# Autodesk Inventor assembly: Left Wheel
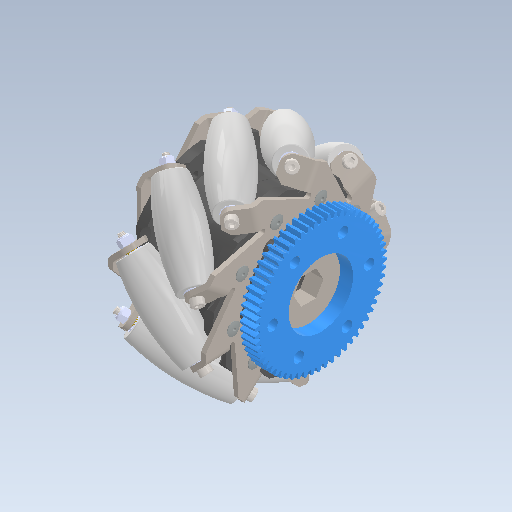
[picture p0: Inventor's stored thumbnail of the model, 512x512]
Saved by Autodesk Inventor 2024.2 (Build 282272000, 272)
## iProperties
Created: 2022-10-15
Part Number: Left Wheel
Document SubType Name: Assembly
Designer: Jason
Author: Jason
## Documents named in this file (4)
- C:\Users\alniles07\Documents\Github\8400_2024_CAD\Left Wheel - Front.iam
- C:\Users\alniles07\Documents\Github\8400_2024_CAD\Left Wheel.ipt
- C:\Users\alniles07\Documents\Github\8400_2024_CAD\Wheel Bearing.ipt
- C:\Users\alniles07\Documents\Github\8400_2024_CAD\FTC Wheel Gear.ipt
## Components (4 placed, 3 different names)
1. Left Wheel:1 — Mate:1, Mate:2, Mate:3, Mate:4, Mate:5, Mate:6, Mate:7
2. Wheel Bearing:1 — Mate:1, Mate:2
3. Wheel Bearing:2 — Mate:3, Mate:4
4. Spur Gear2:1 — Mate:5, Mate:6, Mate:7
## Relationships (7: Mate 7)
- Mate:1: Left Wheel:1 ↔ Wheel Bearing:1
- Mate:2: Left Wheel:1 ↔ Wheel Bearing:1
- Mate:3: Left Wheel:1 ↔ Wheel Bearing:2
- Mate:4: Left Wheel:1 ↔ Wheel Bearing:2
- Mate:5: Left Wheel:1 ↔ Spur Gear2:1
- Mate:6: Left Wheel:1 ↔ Spur Gear2:1
- Mate:7: Left Wheel:1 ↔ Spur Gear2:1
